# Autodesk Inventor assembly: body
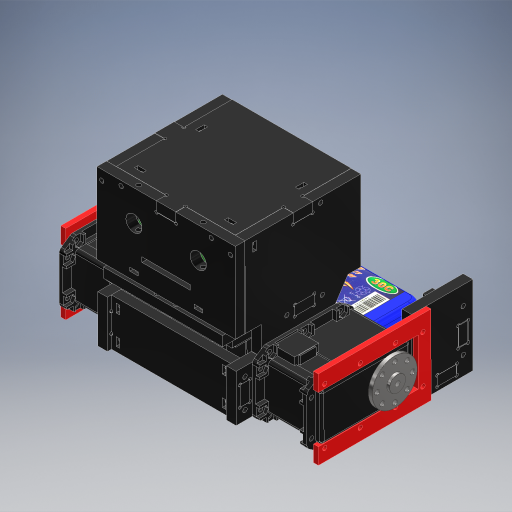
[picture p0: Inventor's stored thumbnail of the model, 512x512]
Saved by Autodesk Inventor 2024 (Build 280153000, 153)
## iProperties
Created: 2024-09-15
Part Number: body
Document SubType Name: Assembly
Designer: msi
Author: msi
## Documents named in this file (18)
- C:\Users\msi\GITHUB\19th_intern_kgh_fight_robot\부품\Upper_body\Body\body.iam
- C:\Users\msi\GITHUB\19th_intern_kgh_fight_robot\부품\Upper_body\Body\connecting plate under body.ipt
- C:\Users\msi\GITHUB\19th_intern_kgh_fight_robot\부품\Upper_body\Body\front of head.ipt
- C:\Users\msi\GITHUB\19th_intern_kgh_fight_robot\부품\Upper_body\Body\overhead.ipt
- C:\Users\msi\GITHUB\19th_intern_kgh_fight_robot\부품\Upper_body\Body\side of head.ipt
- C:\Users\msi\GITHUB\19th_intern_kgh_fight_robot\부품\Upper_body\Body\under the head.ipt
- C:\Users\msi\GITHUB\19th_intern_kgh_fight_robot\부품\Upper_body\Body\battery backplate.ipt
- C:\Users\msi\GITHUB\19th_intern_kgh_fight_robot\부품\Upper_body\Body\battery sideplate.ipt
- C:\Users\msi\GITHUB\19th_intern_kgh_fight_robot\부품\Upper_body\Body\battery bottomplate.ipt
- C:\Users\msi\GITHUB\19th_intern_kgh_fight_robot\부품\ROBOTIS(Inventor 2024 ver.)\다이나믹셀\MX-64T.ipt
- C:\Users\msi\GITHUB\19th_intern_kgh_fight_robot\부품\ROBOTIS(Inventor 2024 ver.)\혼\64-106Horn.ipt
- C:\Users\msi\GITHUB\19th_intern_kgh_fight_robot\부품\Upper_body\Body\waist extension_64.ipt
- C:\Users\msi\GITHUB\19th_intern_kgh_fight_robot\부품\Battery\Enrichpower_2200mAh_11.1V_30C.ipt
- C:\Users\msi\GITHUB\19th_intern_kgh_fight_robot\부품\Circuit\Circuit.ipt
- C:\Users\msi\GITHUB\19th_intern_kgh_fight_robot\부품\Upper_body\Body\body side_battery connection.ipt
- C:\Users\msi\GITHUB\19th_intern_kgh_fight_robot\부품\Upper_body\Body\body front connection.ipt
- body fornt connection.ipt
- C:\Users\msi\GITHUB\19th_intern_kgh_fight_robot\부품\Upper_body\Body\body front connection_fixing part.ipt
## Components (24 placed, 16 different names)
1. connecting plate under body:1 — 삽입:2, 삽입:3, 삽입:4, 삽입:5, 삽입:6, 삽입:7, 삽입:8
2. front of head:1 — 삽입:17, 삽입:18, 삽입:42, 삽입:43
3. overhead:1 — 삽입:42, 삽입:43
4. side of head:1 — 삽입:13, 삽입:14, 삽입:18, 삽입:21
5. under the head:1 — 삽입:19, 삽입:20, 삽입:21, 삽입:40, 삽입:41
6. battery backplate:1 — 삽입:26, 삽입:27, 각도:1, 메이트:6
7. battery sideplate:1 — 삽입:27, 각도:1, 각도:2, 메이트:1, 메이트:4, 삽입:46, 삽입:47
8. battery bottomplate:1 — 각도:2, 메이트:1, 메이트:2, 메이트:3, 메이트:5, 플러쉬:1
9. MX-64T:1 — 삽입:1, 삽입:2, 삽입:3, 삽입:4
10. 64-106Horn:1 — 삽입:1, 삽입:36, 삽입:37
11. MX-64T:2 — 삽입:5, 삽입:6, 삽입:15, 삽입:16, 삽입:38, 삽입:44, 삽입:45, 삽입:56, 삽입:57
12. MX-64T:3 — 삽입:7, 삽입:8, 삽입:13, 삽입:14, 삽입:39, 삽입:48, 삽입:49, 삽입:62, 삽입:63
13. side of head:2 — 삽입:15, 삽입:16, 삽입:17, 삽입:19, 삽입:20
14. battery sideplate:2 — 삽입:26, 메이트:2, 메이트:5, 플러쉬:1, 삽입:50, 삽입:51
15. waist extension_64:1 — 삽입:36, 삽입:37
16. 64-106Horn:2 — 삽입:39
17. 64-106Horn:3 — 삽입:38
18. Enrichpower_2200mAh_11.1V_30C:1 — 메이트:3, 메이트:4, 메이트:6
19. Circuit:1 — 삽입:40, 삽입:41
20. body side_battery connection:1 — 삽입:44, 삽입:45, 삽입:46, 삽입:47
21. body side_battery connection:2 — 삽입:48, 삽입:49, 삽입:50, 삽입:51
22. body fornt connection:1 — 삽입:58, 삽입:59, 삽입:60, 삽입:61
23. body front connection_fixing part:1 — 삽입:56, 삽입:57, 삽입:58, 삽입:59
24. body front connection_fixing part:2 — 삽입:60, 삽입:61, 삽입:62, 삽입:63
## Relationships (52: Insert 43, Mate 6, Angle 2, Flush 1)
- 삽입:1 [Insert]: MX-64T:1 ↔ 64-106Horn:1
- 삽입:2 [Insert]: connecting plate under body:1 ↔ MX-64T:1
- 삽입:3 [Insert]: connecting plate under body:1 ↔ MX-64T:1
- 삽입:4 [Insert]: connecting plate under body:1 ↔ MX-64T:1
- 삽입:5 [Insert]: connecting plate under body:1 ↔ MX-64T:2
- 삽입:6 [Insert]: connecting plate under body:1 ↔ MX-64T:2
- 삽입:7 [Insert]: connecting plate under body:1 ↔ MX-64T:3
- 삽입:8 [Insert]: connecting plate under body:1 ↔ MX-64T:3
- 삽입:13 [Insert]: side of head:1 ↔ MX-64T:3
- 삽입:14 [Insert]: side of head:1 ↔ MX-64T:3
- 삽입:15 [Insert]: MX-64T:2 ↔ side of head:2
- 삽입:16 [Insert]: MX-64T:2 ↔ side of head:2
- 삽입:17 [Insert]: front of head:1 ↔ side of head:2
- 삽입:18 [Insert]: front of head:1 ↔ side of head:1
- 삽입:19 [Insert]: under the head:1 ↔ side of head:2
- 삽입:20 [Insert]: under the head:1 ↔ side of head:2
- 삽입:21 [Insert]: side of head:1 ↔ under the head:1
- 삽입:26 [Insert]: battery backplate:1 ↔ battery sideplate:2
- 삽입:27 [Insert]: battery backplate:1 ↔ battery sideplate:1
- 각도:1 [Angle] (0 deg): battery backplate:1 ↔ battery sideplate:1
- 각도:2 [Angle] (0 deg): battery sideplate:1 ↔ battery bottomplate:1
- 메이트:1 [Mate]: battery sideplate:1 ↔ battery bottomplate:1
- 삽입:36 [Insert]: 64-106Horn:1 ↔ waist extension_64:1
- 삽입:37 [Insert]: 64-106Horn:1 ↔ waist extension_64:1
- 삽입:38 [Insert]: MX-64T:2 ↔ 64-106Horn:3
- 삽입:39 [Insert]: MX-64T:3 ↔ 64-106Horn:2
- 삽입:40 [Insert] (10 mm): under the head:1 ↔ Circuit:1
- 삽입:41 [Insert] (10 mm): under the head:1 ↔ Circuit:1
- 삽입:42 [Insert]: front of head:1 ↔ overhead:1
- 삽입:43 [Insert]: front of head:1 ↔ overhead:1
- 메이트:2 [Mate]: battery bottomplate:1 ↔ battery sideplate:2
- 메이트:3 [Mate]: battery bottomplate:1 ↔ Enrichpower_2200mAh_11.1V_30C:1
- 메이트:4 [Mate] (17 mm): battery sideplate:1 ↔ Enrichpower_2200mAh_11.1V_30C:1
- 메이트:5 [Mate]: battery bottomplate:1 ↔ battery sideplate:2
- 플러쉬:1 [Flush]: battery bottomplate:1 ↔ battery sideplate:2
- 메이트:6 [Mate]: battery backplate:1 ↔ Enrichpower_2200mAh_11.1V_30C:1
- 삽입:44 [Insert]: MX-64T:2 ↔ body side_battery connection:1
- 삽입:45 [Insert]: MX-64T:2 ↔ body side_battery connection:1
- 삽입:46 [Insert]: battery sideplate:1 ↔ body side_battery connection:1
- 삽입:47 [Insert]: battery sideplate:1 ↔ body side_battery connection:1
- 삽입:48 [Insert]: MX-64T:3 ↔ body side_battery connection:2
- 삽입:49 [Insert]: MX-64T:3 ↔ body side_battery connection:2
- 삽입:50 [Insert]: battery sideplate:2 ↔ body side_battery connection:2
- 삽입:51 [Insert]: battery sideplate:2 ↔ body side_battery connection:2
- 삽입:56 [Insert]: MX-64T:2 ↔ body front connection_fixing part:1
- 삽입:57 [Insert]: MX-64T:2 ↔ body front connection_fixing part:1
- 삽입:58 [Insert]: body fornt connection:1 ↔ body front connection_fixing part:1
- 삽입:59 [Insert]: body fornt connection:1 ↔ body front connection_fixing part:1
- 삽입:60 [Insert]: body fornt connection:1 ↔ body front connection_fixing part:2
- 삽입:61 [Insert]: body fornt connection:1 ↔ body front connection_fixing part:2
- 삽입:62 [Insert]: MX-64T:3 ↔ body front connection_fixing part:2
- 삽입:63 [Insert]: MX-64T:3 ↔ body front connection_fixing part:2
